# Autodesk Inventor assembly: Stereo Camera Holder
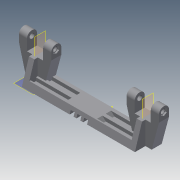
[picture p0: Inventor's stored thumbnail of the model, 180x180]
Saved by Autodesk Inventor 2018 (Build 220112000, 112)
## iProperties
Created: 2018-11-16
Part Number: Stereo Camera Holder
Document SubType Name: Assembly
Designer: Micah
Author: Micah
## Documents named in this file (3)
- C:\Users\Micah\OneDrive\Fall 2018\Intro to Robotics\Stereo Camera Holder.iam
- C:\Users\Micah\OneDrive\Fall 2018\Intro to Robotics\Camera Holder.ipt
- C:\Users\Micah\OneDrive\Fall 2018\Intro to Robotics\Connecting arm.ipt
## Components (3 placed, 2 different names)
1. Camera Holder:1 — Flush:1, Mate:1, Flush:2
2. Camera Holder:2 — Flush:1, Mate:1
3. Connecting arm:1 — Flush:2
## Relationships (3: Flush 2, Mate 1)
- Flush:1 (101.6 mm): Camera Holder:1 ↔ Camera Holder:2
- Mate:1: Camera Holder:1 ↔ Camera Holder:2
- Flush:2: Camera Holder:1 ↔ Connecting arm:1
